# Autodesk Inventor assembly: Protjeto Final
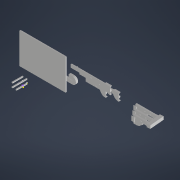
[picture p0: Inventor's stored thumbnail of the model, 180x180]
Saved by Autodesk Inventor 2022 (Build 260153000, 153)
## iProperties
Created: 2023-05-10
Part Number: Protjeto Final
Document SubType Name: Assembly
Designer: nevin
Author: nevin
## Documents named in this file (13)
- G:\My Drive\Faculdade\Trabalhos\Desenho e Print 3D\Marbles project\Protjeto Final.iam
- G:\My Drive\Faculdade\Trabalhos\Desenho e Print 3D\Marbles project\Base.ipt
- G:\My Drive\Faculdade\Trabalhos\Desenho e Print 3D\Marbles project\Pega uma e libera superior.ipt
- G:\My Drive\Faculdade\Trabalhos\Desenho e Print 3D\Marbles project\Pega uma e libera.ipt
- G:\My Drive\Faculdade\Trabalhos\Desenho e Print 3D\Marbles project\Receptor pequeno.ipt
- G:\My Drive\Faculdade\Trabalhos\Desenho e Print 3D\Marbles project\Receptor.ipt
- G:\My Drive\Faculdade\Trabalhos\Desenho e Print 3D\Marbles project\Trilho 5 minutos.ipt
- G:\My Drive\Faculdade\Trabalhos\Desenho e Print 3D\Marbles project\Trilho 60 minutos  - 12 horas.ipt
- G:\My Drive\Faculdade\Trabalhos\Desenho e Print 3D\Marbles project\Troca de sentido.ipt
- G:\My Drive\Faculdade\Trabalhos\Desenho e Print 3D\Marbles project\Sustentação Trilhos fixos.ipt
- G:\My Drive\Faculdade\Trabalhos\Desenho e Print 3D\Marbles project\Box de reinício.ipt
- G:\My Drive\Faculdade\Trabalhos\Desenho e Print 3D\Marbles project\Conector superior para giro.ipt
- G:\My Drive\Faculdade\Trabalhos\Desenho e Print 3D\Marbles project\Libera todas.ipt
## Components (16 placed, 12 different names)
1. Base:1
2. Pega uma e libera superior:1 — Inserir:4, Alinhado:1, Alinhado:4, Inserir:11
3. Receptor pequeno:1 — Alinhado:4, Inserir:12
4. Receptor:1 — Inserir:1
5. Trilho 5 minutos:1 — Inserir:1
6. Trilho 60 minutos  - 12 horas:1 — Inserir:13
7. Troca de sentido:1 — Inserir:5
8. Receptor:2 — Inserir:13
9. Trilho 60 minutos  - 12 horas:2 — Inserir:2
10. Receptor:3 — Inserir:2
11. Pega uma e libera:2 — Inserir:7, Alinhado:2, Alinhado:5, Inserir:12
12. Receptor pequeno:2 — Alinhado:5, Inserir:11
13. Sustentação Trilhos fixos:1
14. Box de reinício:1 — Inserir:4, Inserir:6, Inserir:7, Alinhado:1, Alinhado:2, Alinhado:3
15. Conector superior para giro:1 — Inserir:5
16. Libera todas:1 — Inserir:6, Alinhado:3
## Relationships (14: Insert 9, Flush 5)
- Inserir:1: Receptor:1 ↔ Trilho 5 minutos:1
- Inserir:2: Trilho 60 minutos  - 12 horas:2 ↔ Receptor:3
- Inserir:4: Pega uma e libera superior:1 ↔ Box de reinício:1
- Inserir:5: Troca de sentido:1 ↔ Conector superior para giro:1
- Inserir:6: Box de reinício:1 ↔ Libera todas:1
- Inserir:7: Pega uma e libera:2 ↔ Box de reinício:1
- Alinhado:1 [Flush]: Pega uma e libera superior:1 ↔ Box de reinício:1
- Alinhado:2 [Flush]: Pega uma e libera:2 ↔ Box de reinício:1
- Alinhado:3 [Flush]: Box de reinício:1 ↔ Libera todas:1
- Alinhado:4 [Flush]: Pega uma e libera superior:1 ↔ Receptor pequeno:1
- Alinhado:5 [Flush]: Pega uma e libera:2 ↔ Receptor pequeno:2
- Inserir:11 (9 mm): Pega uma e libera superior:1 ↔ Receptor pequeno:2
- Inserir:12 (9 mm): Receptor pequeno:1 ↔ Pega uma e libera:2
- Inserir:13: Trilho 60 minutos  - 12 horas:1 ↔ Receptor:2
## Named parameters: Diâmetro_esfera = 18 mm
